# Autodesk Inventor assembly: palec
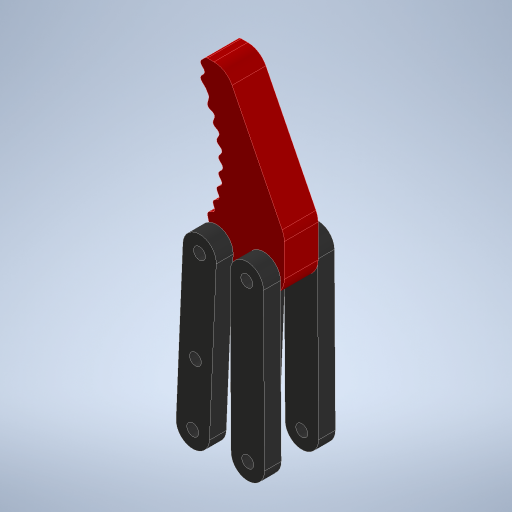
[picture p0: Inventor's stored thumbnail of the model, 512x512]
Saved by Autodesk Inventor 2023 (Build 270158000, 158)
## iProperties
Created: 2023-06-03
Part Number: palec
Document SubType Name: Assembly
Designer: komputer
Author: komputer
## iProperties of the stored document MemberDocs/xAaaaqrdaAaaaaaaaAaaaa2jiAh
Part Number: palec
Document SubType Name: Zespół
Designer: Kamil
Author: Kamil
## Documents named in this file (5)
- C:\Users\Kamil\Desktop\KONARM_2\chwytak\palec.iam
- C:\Users\Kamil\Desktop\KONARM_2\chwytak\GripperClaw.ipt
- C:\Users\Kamil\Desktop\KONARM_2\chwytak\Arm.ipt
- C:\Users\Kamil\Desktop\KONARM_2\chwytak\ArmOuter.ipt
- C:\Users\Kamil\Desktop\KONARM_2\chwytak\palec_SUB.ipt
## Components (5 placed, 3 different names)
1. GripperClaw:1 — Zestawiające:10, Zestawiające:11, Zestawiające:12, Zestawiające:13, Zestawiające:15, Zestawiające:16, Zestawiające:17, Zestawiające:18
2. Arm:1 — Zestawiające:10, Zestawiające:13, Zestawiające:14
3. Arm:2 — Zestawiające:11, Zestawiające:12, Zestawiające:14
4. ArmOuter:1 — Zestawiające:15, Zestawiające:17, Zestawiające:19
5. ArmOuter:2 — Zestawiające:16, Zestawiające:18, Zestawiające:19
## Relationships (10: Mate 10)
- Zestawiające:10 [Mate] (0.5 mm): GripperClaw:1 ↔ Arm:1
- Zestawiające:11 [Mate] (0.5 mm): GripperClaw:1 ↔ Arm:2
- Zestawiające:12 [Mate]: GripperClaw:1 ↔ Arm:2
- Zestawiające:13 [Mate]: GripperClaw:1 ↔ Arm:1
- Zestawiające:14 [Mate]: Arm:1 ↔ Arm:2
- Zestawiające:15 [Mate] (0.5 mm): GripperClaw:1 ↔ ArmOuter:1
- Zestawiające:16 [Mate] (0.5 mm): GripperClaw:1 ↔ ArmOuter:2
- Zestawiające:17 [Mate]: GripperClaw:1 ↔ ArmOuter:1
- Zestawiające:18 [Mate]: GripperClaw:1 ↔ ArmOuter:2
- Zestawiające:19 [Mate]: ArmOuter:1 ↔ ArmOuter:2
